# Autodesk Inventor assembly: ASY MSC 203 RIGHT BOARD
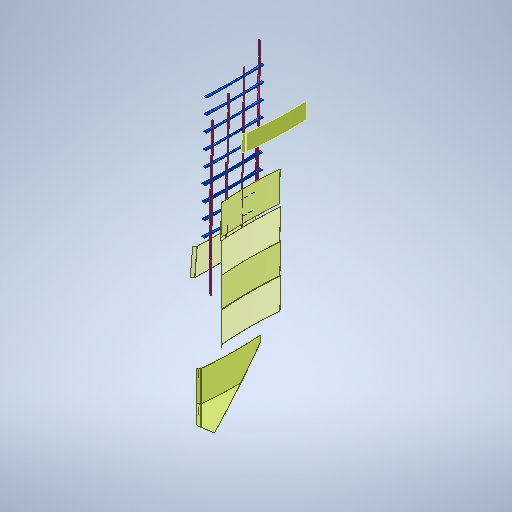
[picture p0: Inventor's stored thumbnail of the model, 512x512]
Saved by Autodesk Inventor 2025 (Build 290162010, 162A)
## iProperties
Created: 2024-07-22
Part Number: ASY MSC 203 RIGHT BOARD
Document SubType Name: Assembly
Designer: pokla
Author: pokla
## Documents named in this file (10)
- C:\Users\admin\YandexDisk-badmisterfox\домашниий пк\Inventor\Manturovo\Manturovo_Se-clar\ASY MSC 203 RIGHT BOARD.iam
- C:\Users\admin\YandexDisk-badmisterfox\домашниий пк\Inventor\Manturovo\Manturovo_Se-clar\MSC 052 rib board.ipt
- C:\Users\admin\YandexDisk-badmisterfox\домашниий пк\Inventor\Manturovo\Manturovo_Se-clar\MSC 024 sheet board main.ipt
- C:\Users\admin\YandexDisk-badmisterfox\домашниий пк\Inventor\Manturovo\Manturovo_Se-clar\MSC 023 sheet board.ipt
- C:\Users\admin\YandexDisk-badmisterfox\домашниий пк\Inventor\Manturovo\Manturovo_Se-clar\MSC 025.2 sheet board withers.ipt
- C:\Users\admin\YandexDisk-badmisterfox\домашниий пк\Inventor\Manturovo\Manturovo_Se-clar\MSC 063 stringer BOARD  #.ipt
- C:\Users\admin\YandexDisk-badmisterfox\домашниий пк\Inventor\Manturovo\Manturovo_Se-clar\MSC 064 stringer BOARD  ##.ipt
- C:\Users\admin\YandexDisk-badmisterfox\домашниий пк\Inventor\Manturovo\Manturovo_Se-clar\MSC 027.2 sheet board withers 4.ipt
- C:\Users\admin\YandexDisk-badmisterfox\домашниий пк\Inventor\Manturovo\Manturovo_Se-clar\MSC 065 stringer BOARD  ###.ipt
- C:\Users\admin\YandexDisk-badmisterfox\домашниий пк\Inventor\Manturovo\Manturovo_Se-clar\MSC 065 stringer BOARD  ####.ipt
## Components (46 placed, 10 different names)
1. MSC 023 sheet board.ipt:2 — Flush:6
2. MSC 024 sheet board main.ipt:10
3. MSC 024 sheet board main.ipt:9
4. MSC 024 sheet board main.ipt:8
5. MSC 024 sheet board main.ipt:7
6. MSC 024 sheet board main.ipt:6
7. MSC 025.2 sheet board withers:1 — Rigid:57
8. MSC 027.2 sheet board withers 4:1 — Rigid:57
9. MSC 052 rib board.ipt:1 — Rigid:43, Flush:3, Rigid:61, Flush:4
10. MSC 052 rib board.ipt:4 — Rigid:44, Rigid:45
11. MSC 052 rib board:3 — Rigid:62
12. MSC 063 stringer BOARD  #:1 — Rigid:43, Rigid:44, Rigid:53, Flush:5
13. MSC 064 stringer BOARD  ##:1 — Rigid:45, Rigid:58
14. MSC 065 stringer BOARD  ###:1 — Rigid:49, Rigid:52, Rigid:55
15. MSC 065 stringer BOARD  ####:1 — Rigid:50, Rigid:59, Rigid:60
16. MSC 065 stringer BOARD  ####:2 — Rigid:59
17. MSC 065 stringer BOARD  ###:2 — Rigid:52, Rigid:61
18. MSC 065 stringer BOARD  ####:3 — Rigid:60
19. MSC 065 stringer BOARD  ###:3 — Rigid:55
20. MSC 064 stringer BOARD  ##:2 — Rigid:58
21. MSC 063 stringer BOARD  #:2 — Rigid:53, Rigid:62
22. MSC 065 stringer BOARD  ####:4
23. MSC 065 stringer BOARD  ###:4
24. MSC 064 stringer BOARD  ##:3
25. MSC 063 stringer BOARD  #:3
26. MSC 065 stringer BOARD  ####:5
27. MSC 065 stringer BOARD  ###:5
28. MSC 064 stringer BOARD  ##:4
29. MSC 063 stringer BOARD  #:4
30. MSC 065 stringer BOARD  ####:6
31. MSC 065 stringer BOARD  ###:6
32. MSC 064 stringer BOARD  ##:5
33. MSC 063 stringer BOARD  #:5
34. MSC 065 stringer BOARD  ####:7
35. MSC 065 stringer BOARD  ###:7
36. MSC 064 stringer BOARD  ##:6
37. MSC 063 stringer BOARD  #:6
38. MSC 052 rib board:5 — Rigid:49, Rigid:50
39. MSC 052 rib board:6
40. MSC 052 rib board:7
41. MSC 052 rib board:8
42. MSC 052 rib board:9
43. MSC 052 rib board:10
44. MSC 052 rib board:11
45. MSC 052 rib board:12
46. MSC 052 rib board:13 — Flush:6
## Component patterns: (5 elements, first: MSC 065 stringer BOARD  ####:3 + MSC 065 stringer BOARD  ###:3 + MSC 064 stringer BOARD  ##:2 + MSC 063 stringer BOARD  #:2), (9 elements, first: MSC 052 rib board:5)
## Relationships (18: WeldJoint 14, Flush 4)
- Rigid:43 [WeldJoint] (2 mm): MSC 052 rib board.ipt:1 ↔ MSC 063 stringer BOARD  #:1
- Rigid:44 [WeldJoint] (2 mm): MSC 052 rib board.ipt:4 ↔ MSC 063 stringer BOARD  #:1
- Rigid:45 [WeldJoint] (2 mm): MSC 052 rib board.ipt:4 ↔ MSC 064 stringer BOARD  ##:1
- Rigid:49 [WeldJoint] (2 mm): MSC 065 stringer BOARD  ###:1 ↔ MSC 052 rib board:5
- Rigid:50 [WeldJoint] (2 mm): MSC 065 stringer BOARD  ####:1 ↔ MSC 052 rib board:5
- Rigid:52 [WeldJoint]: MSC 065 stringer BOARD  ###:1 ↔ MSC 065 stringer BOARD  ###:2
- Rigid:53 [WeldJoint]: MSC 063 stringer BOARD  #:1 ↔ MSC 063 stringer BOARD  #:2
- Rigid:55 [WeldJoint]: MSC 065 stringer BOARD  ###:1 ↔ MSC 065 stringer BOARD  ###:3
- Rigid:57 [WeldJoint]: MSC 025.2 sheet board withers:1 ↔ MSC 027.2 sheet board withers 4:1
- Flush:3: MSC 052 rib board.ipt:1
- Rigid:58 [WeldJoint]: MSC 064 stringer BOARD  ##:1 ↔ MSC 064 stringer BOARD  ##:2
- Rigid:59 [WeldJoint]: MSC 065 stringer BOARD  ####:1 ↔ MSC 065 stringer BOARD  ####:2
- Rigid:60 [WeldJoint]: MSC 065 stringer BOARD  ####:1 ↔ MSC 065 stringer BOARD  ####:3
- Rigid:61 [WeldJoint]: MSC 052 rib board.ipt:1 ↔ MSC 065 stringer BOARD  ###:2
- Rigid:62 [WeldJoint]: MSC 052 rib board:3 ↔ MSC 063 stringer BOARD  #:2
- Flush:4: MSC 052 rib board.ipt:1
- Flush:5: MSC 063 stringer BOARD  #:1
- Flush:6 (-304 mm): MSC 023 sheet board.ipt:2 ↔ MSC 052 rib board:13
